# Autodesk Inventor assembly: Assembly3manifold
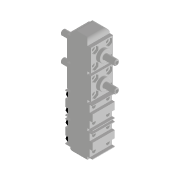
[picture p0: Inventor's stored thumbnail of the model, 180x180]
Saved by Autodesk Inventor 2020 (Build 240168000, 168)
## iProperties
Created: 2020-09-03
Part Number: Assembly3manifold
Document SubType Name: Assembly
Designer: Admin
Author: Admin
## Documents named in this file (5)
- C:\PFE\Project_github\YFA-Project_python_interface\3D models\Assembly3manifold.iam
- C:\PFE\Project_github\YFA-Project_python_interface\3D models\to_print_30_06\MANIFOLD.ipt
- C:\PFE\Project_github\YFA-Project_python_interface\3D models\to_print_30_06\INTERFACE_MANIFOLD.ipt
- C:\PFE\Project_github\YFA-Project_python_interface\3D models\to_print_30_06\INTERFACE_MANIFOLD_KORK.ipt
- C:\PFE\Project_github\YFA-Project_python_interface\3D models\to_print_11_08\NUT.ipt
## Components (25 placed, 4 different names)
1. MANIFOLD:1 — Mate:9, Mate:10, Mate:11, Mate:12, Flush:1, Flush:2, Flush:3, Flush:4, Mate:13, Mate:14, Mate:15, Mate:16, Mate:17, Mate:18, Mate:19, Mate:20, Mate:21, Mate:22, Mate:23, Mate:24, Mate:25, Mate:26, Mate:27, Mate:28
2. INTERFACE_MANIFOLD:1 — Mate:9, Flush:1, Mate:25, Mate:29, Mate:30, Mate:31, Mate:43
3. INTERFACE_MANIFOLD:2 — Mate:10, Flush:2, Mate:26, Mate:32, Mate:33, Mate:41, Mate:44
4. INTERFACE_MANIFOLD:3 — Mate:11, Flush:3, Mate:24
5. INTERFACE_MANIFOLD:4 — Mate:12, Flush:4, Mate:23
6. INTERFACE_MANIFOLD_KORK:1 — Mate:15, Mate:16, Mate:27, Mate:38, Mate:39, Mate:40, Mate:42
7. INTERFACE_MANIFOLD_KORK:2 — Mate:13, Mate:14, Mate:28, Mate:34, Mate:35, Mate:36, Mate:37
8. INTERFACE_MANIFOLD_KORK:3 — Mate:17, Mate:18, Mate:22
9. INTERFACE_MANIFOLD_KORK:4 — Mate:19, Mate:20, Mate:21
10. NUT:1 — Mate:41
11. NUT:2 — Mate:40
12. NUT:3 — Mate:34
13. NUT:4 — Mate:33
14. NUT:5 — Mate:31
15. NUT:6 — Mate:38
16. NUT:7 — Mate:39
17. NUT:8 — Mate:43
18. NUT:9 — Mate:44
19. NUT:10 — Mate:42
20. NUT:11 — Mate:37
21. NUT:12 — Mate:36
22. NUT:13 — Mate:35
23. NUT:14 — Mate:30
24. NUT:15 — Mate:29
25. NUT:16 — Mate:32
## Relationships (40: Mate 36, Flush 4)
- Mate:9: MANIFOLD:1 ↔ INTERFACE_MANIFOLD:1
- Mate:10: MANIFOLD:1 ↔ INTERFACE_MANIFOLD:2
- Mate:11: MANIFOLD:1 ↔ INTERFACE_MANIFOLD:3
- Mate:12: MANIFOLD:1 ↔ INTERFACE_MANIFOLD:4
- Flush:1: MANIFOLD:1 ↔ INTERFACE_MANIFOLD:1
- Flush:2: MANIFOLD:1 ↔ INTERFACE_MANIFOLD:2
- Flush:3: MANIFOLD:1 ↔ INTERFACE_MANIFOLD:3
- Flush:4: MANIFOLD:1 ↔ INTERFACE_MANIFOLD:4
- Mate:13: MANIFOLD:1 ↔ INTERFACE_MANIFOLD_KORK:2
- Mate:14: MANIFOLD:1 ↔ INTERFACE_MANIFOLD_KORK:2
- Mate:15: MANIFOLD:1 ↔ INTERFACE_MANIFOLD_KORK:1
- Mate:16: MANIFOLD:1 ↔ INTERFACE_MANIFOLD_KORK:1
- Mate:17: MANIFOLD:1 ↔ INTERFACE_MANIFOLD_KORK:3
- Mate:18: MANIFOLD:1 ↔ INTERFACE_MANIFOLD_KORK:3
- Mate:19: MANIFOLD:1 ↔ INTERFACE_MANIFOLD_KORK:4
- Mate:20: MANIFOLD:1 ↔ INTERFACE_MANIFOLD_KORK:4
- Mate:21: MANIFOLD:1 ↔ INTERFACE_MANIFOLD_KORK:4
- Mate:22: MANIFOLD:1 ↔ INTERFACE_MANIFOLD_KORK:3
- Mate:23: MANIFOLD:1 ↔ INTERFACE_MANIFOLD:4
- Mate:24: MANIFOLD:1 ↔ INTERFACE_MANIFOLD:3
- Mate:25: MANIFOLD:1 ↔ INTERFACE_MANIFOLD:1
- Mate:26: MANIFOLD:1 ↔ INTERFACE_MANIFOLD:2
- Mate:27: MANIFOLD:1 ↔ INTERFACE_MANIFOLD_KORK:1
- Mate:28: MANIFOLD:1 ↔ INTERFACE_MANIFOLD_KORK:2
- Mate:29: INTERFACE_MANIFOLD:1 ↔ NUT:15
- Mate:30: INTERFACE_MANIFOLD:1 ↔ NUT:14
- Mate:31: INTERFACE_MANIFOLD:1 ↔ NUT:5
- Mate:32: INTERFACE_MANIFOLD:2 ↔ NUT:16
- Mate:33: INTERFACE_MANIFOLD:2 ↔ NUT:4
- Mate:34: INTERFACE_MANIFOLD_KORK:2 ↔ NUT:3
- Mate:35: INTERFACE_MANIFOLD_KORK:2 ↔ NUT:13
- Mate:36: INTERFACE_MANIFOLD_KORK:2 ↔ NUT:12
- Mate:37: INTERFACE_MANIFOLD_KORK:2 ↔ NUT:11
- Mate:38: INTERFACE_MANIFOLD_KORK:1 ↔ NUT:6
- Mate:39: INTERFACE_MANIFOLD_KORK:1 ↔ NUT:7
- Mate:40: INTERFACE_MANIFOLD_KORK:1 ↔ NUT:2
- Mate:41: INTERFACE_MANIFOLD:2 ↔ NUT:1
- Mate:42: INTERFACE_MANIFOLD_KORK:1 ↔ NUT:10
- Mate:43: INTERFACE_MANIFOLD:1 ↔ NUT:8
- Mate:44: INTERFACE_MANIFOLD:2 ↔ NUT:9
